# Autodesk Inventor assembly: ASSEMBLY_Blade
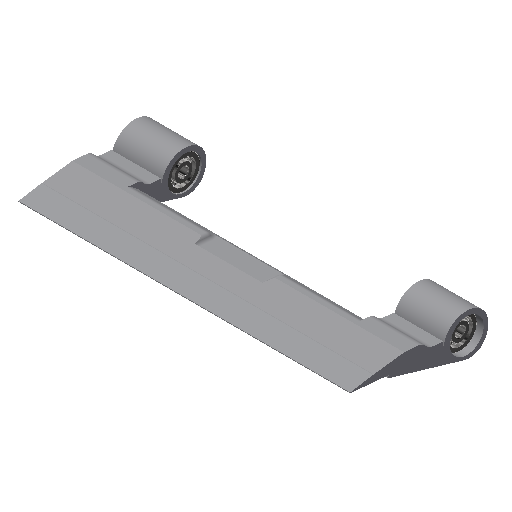
[picture p0: Inventor's stored thumbnail of the model, 512x512]
Saved by Autodesk Inventor 2026.1 (Build 301233000, 233)
## iProperties
Created: 2016-06-10
Part Number: ASSEMBLY_Blade
Material: Ogólny
Document SubType Name: Assembly
Designer: Andrzej
Mass: 10.1599 g
Surface Area: 107.992 cm^2
Volume: 10.1599 cm^3
Density: 1 g/cm^3
Author: Andrzej
## Documents named in this file (5)
- C:\Users\Andrzej\OneDrive\_DRIVE_SYNCH_FILES\__ BYTECHLAB PROJECTS\MLTDIS - Mini Sumo Robot - Bullet XT\MCAD\1_REV1\ASSEMBLY_MAIN_REVA\ASSEMBLY_Blade.iam
- C:\Users\Andrzej\OneDrive\_DRIVE_SYNCH_FILES\__ BYTECHLAB PROJECTS\MLTDIS - Mini Sumo Robot - Bullet XT\MCAD\1_REV1\__COTS_PARTS\COTS_SKF_623_RS_285-0790_Bearing.ipt
- C:\Users\Andrzej\OneDrive\_DRIVE_SYNCH_FILES\__ BYTECHLAB PROJECTS\MLTDIS - Mini Sumo Robot - Bullet XT\MCAD\1_REV1\ASSEMBLY_MAIN_REVA\3DP_PLA_Front_blade.ipt
- C:\Users\Andrzej\OneDrive\_DRIVE_SYNCH_FILES\__ BYTECHLAB PROJECTS\MLTDIS - Mini Sumo Robot - Bullet XT\MCAD\1_REV1\ASSEMBLY_MAIN_REVA\3DP_PLA_Front_blade_hinge.ipt
- C:\Users\Andrzej\OneDrive\_DRIVE_SYNCH_FILES\__ BYTECHLAB PROJECTS\MLTDIS - Mini Sumo Robot - Bullet XT\MCAD\1_REV1\ASSEMBLY_MAIN_REVA\3DP_PLA_Front_blade_hinge_mir.ipt
## Components (7 placed, 4 different names)
1. COTS_SKF_623_RS_285-0790_Bearing:1 — Zestawiający:5, Styczny:3
2. COTS_SKF_623_RS_285-0790_Bearing:2 — Zestawiający:6, Styczny:4
3. COTS_SKF_623_RS_285-0790_Bearing:3 — Zestawiający:8, Styczny:1
4. COTS_SKF_623_RS_285-0790_Bearing:4 — Zestawiający:7, Styczny:2
5. 3DP_PLA_Front_blade:1 — Równoległy:1, Równoległy:2, Zestawiający:9, Zestawiający:10, Zestawiający:11, Zestawiający:12
6. 3DP_PLA_Front_blade_hinge:1 — Zestawiający:6, Zestawiający:8, Styczny:1, Styczny:4, Równoległy:2, Zestawiający:10, Zestawiający:11
7. 3DP_PLA_Front_blade_hinge_mir:1 — Zestawiający:5, Zestawiający:7, Styczny:2, Styczny:3, Równoległy:1, Zestawiający:9, Zestawiający:12
## Relationships (14: Mate 8, Tangent 4, Flush 2)
- Zestawiający:5 [Mate]: COTS_SKF_623_RS_285-0790_Bearing:1 ↔ 3DP_PLA_Front_blade_hinge_mir:1
- Zestawiający:6 [Mate]: COTS_SKF_623_RS_285-0790_Bearing:2 ↔ 3DP_PLA_Front_blade_hinge:1
- Zestawiający:7 [Mate]: COTS_SKF_623_RS_285-0790_Bearing:4 ↔ 3DP_PLA_Front_blade_hinge_mir:1
- Zestawiający:8 [Mate]: COTS_SKF_623_RS_285-0790_Bearing:3 ↔ 3DP_PLA_Front_blade_hinge:1
- Styczny:1 [Tangent]: COTS_SKF_623_RS_285-0790_Bearing:3 ↔ 3DP_PLA_Front_blade_hinge:1
- Styczny:2 [Tangent]: COTS_SKF_623_RS_285-0790_Bearing:4 ↔ 3DP_PLA_Front_blade_hinge_mir:1
- Styczny:3 [Tangent]: COTS_SKF_623_RS_285-0790_Bearing:1 ↔ 3DP_PLA_Front_blade_hinge_mir:1
- Styczny:4 [Tangent]: COTS_SKF_623_RS_285-0790_Bearing:2 ↔ 3DP_PLA_Front_blade_hinge:1
- Równoległy:1 [Flush]: 3DP_PLA_Front_blade:1 ↔ 3DP_PLA_Front_blade_hinge_mir:1
- Równoległy:2 [Flush]: 3DP_PLA_Front_blade:1 ↔ 3DP_PLA_Front_blade_hinge:1
- Zestawiający:9 [Mate]: 3DP_PLA_Front_blade:1 ↔ 3DP_PLA_Front_blade_hinge_mir:1
- Zestawiający:10 [Mate]: 3DP_PLA_Front_blade:1 ↔ 3DP_PLA_Front_blade_hinge:1
- Zestawiający:11 [Mate]: 3DP_PLA_Front_blade:1 ↔ 3DP_PLA_Front_blade_hinge:1
- Zestawiający:12 [Mate]: 3DP_PLA_Front_blade:1 ↔ 3DP_PLA_Front_blade_hinge_mir:1
